# Autodesk Inventor assembly: MEGA 2560 PRO (EMBED)
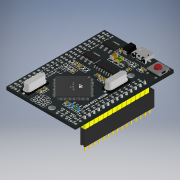
[picture p0: Inventor's stored thumbnail of the model, 180x180]
Saved by Autodesk Inventor 2020 (Build 240168000, 168)
## iProperties
Company: Unknown
Created: 2019-01-02
Part Number: MEGA 2560 PRO (EMBED)
Description: Unknown
Document SubType Name: Assembly
Designer: Ivan
Sending System: DEX
Preprocessor: ST-DEVELOPER v16.7
Title: MEGA 2560 PRO (EMBED)
Author: Unknown
## Documents named in this file (19)
- C:\!projects\DASH_\3D\omni_platorm\step\mega\MEGA 2560 PRO (EMBED).iam
- C:\!projects\DASH_\3D\omni_platorm\step\mega\Mega 2560 Pro - Board.ipt
- C:\!projects\DASH_\3D\omni_platorm\step\mega\SOT223-3.ipt
- C:\!projects\DASH_\3D\omni_platorm\step\mega\ATmega2560-16AU.ipt
- C:\!projects\DASH_\3D\omni_platorm\step\mega\SOIC -16.ipt
- C:\!projects\DASH_\3D\omni_platorm\step\mega\Crystal Oscillator (SMD).ipt
- C:\!projects\DASH_\3D\omni_platorm\step\mega\1206 Capacitor.ipt
- C:\!projects\DASH_\3D\omni_platorm\step\mega\Fuse (1206) - Green.ipt
- C:\!projects\DASH_\3D\omni_platorm\step\mega\Diode - SMD - DO-214AC.ipt
- C:\!projects\DASH_\3D\omni_platorm\step\mega\USB - Micro.ipt
- C:\!projects\DASH_\3D\omni_platorm\step\mega\0603 Capacitor.ipt
- C:\!projects\DASH_\3D\omni_platorm\step\mega\0603 Resistor.ipt
- C:\!projects\DASH_\3D\omni_platorm\step\mega\LED - 0603 - Blue.ipt
- C:\!projects\DASH_\3D\omni_platorm\step\mega\LED_-_Vishay_-_6063_-_Green.ipt
- C:\!projects\DASH_\3D\omni_platorm\step\mega\1206 Fuse.ipt
- C:\!projects\DASH_\3D\omni_platorm\step\mega\SWT-32.ipt
- C:\!projects\DASH_\3D\omni_platorm\step\PLS-14\PLS-14.iam
- C:\!projects\DASH_\3D\omni_platorm\step\mega\mega_switchboard.ipt
- C:\!projects\DASH_\3D\omni_platorm\step\PLS_15\PBS-15.ipt
## Components (46 placed, 18 different names)
1. Mega 2560 Pro - Board — Вставка:1, Угол:1, Вставка:2, Заподлицо:1
2. SOT223-3
3. SOT223-3:1
4. ATmega2560-16AU
5. SOIC -16
6. Crystal Oscillator (SMD)
7. Crystal Oscillator (SMD):1
8. 1206 Capacitor
9. Fuse (1206) - Green
10. Diode - SMD - DO-214AC
11. USB - Micro
12. 0603 Capacitor
13. 0603 Capacitor:1
14. 0603 Capacitor:2
15. 0603 Capacitor:3
16. 0603 Capacitor:4
17. 0603 Capacitor:5
18. 0603 Capacitor:6
19. 0603 Capacitor:7
20. 0603 Capacitor:8
21. 0603 Capacitor:9
22. 0603 Capacitor:10
23. 0603 Capacitor:11
24. 0603 Capacitor:12
25. 0603 Capacitor:13
26. 0603 Resistor
27. 0603 Resistor:1
28. 0603 Resistor:2
29. 0603 Resistor:3
30. 0603 Resistor:4
31. 0603 Resistor:5
32. 0603 Resistor:6
33. 0603 Resistor:7
34. 0603 Resistor:8
35. 0603 Resistor:9
36. 0603 Resistor:10
37. 0603 Resistor:11
38. LED - 0603 - Blue
39. LED_-_Vishay_-_6063_-_Green
40. LED - 0603 - Blue:1
41. 1206 Fuse
42. SWT-32
43. LED - 0603 - Blue:2
44. PLS-14:1 [sub-assembly] — Вставка:1, Угол:1, Совмещение:1, Совмещение:2, Совмещение:3
45. mega_switchboard:1 — Вставка:2, Заподлицо:1
46. PBS-15:1 — Совмещение:1, Совмещение:2, Совмещение:3
## Relationships (7: Mate 3, Insert 2, Angle 1, Flush 1)
- Вставка:1 [Insert] (-10.075 mm): Mega 2560 Pro - Board ↔ PLS-14:1
- Угол:1 [Angle] (0 deg): Mega 2560 Pro - Board ↔ PLS-14:1
- Вставка:2 [Insert] (8.5 mm): Mega 2560 Pro - Board ↔ mega_switchboard:1
- Заподлицо:1 [Flush]: Mega 2560 Pro - Board ↔ mega_switchboard:1
- Совмещение:1 [Mate]: PLS-14:1 ↔ PBS-15:1
- Совмещение:2 [Mate]: PLS-14:1 ↔ PBS-15:1
- Совмещение:3 [Mate]: PLS-14:1 ↔ PBS-15:1
